# Autodesk Inventor assembly: A2017_T4_11
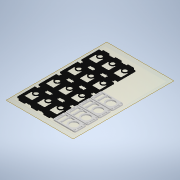
[picture p0: Inventor's stored thumbnail of the model, 180x180]
Saved by Autodesk Inventor 2020 (Build 240168000, 168)
## iProperties
Created: 2021-08-27
Part Number: A2017_T4_11
Document SubType Name: Assembly
Designer: Masato
Author: Masato
## Documents named in this file (4)
- C:\Inventor\SUSTAINA-OP\Cam\A2017_T4_11.iam
- C:\Inventor\SUSTAINA-OP\Cam\DisposableBoard.ipt
- C:\Inventor\SUSTAINA-OP\UpperBody\Trunk\Trunk_neck_frame.ipt
- C:\Inventor\SUSTAINA-OP\UpperBody\Trunk\Trunk_servo_bottom_frame.ipt
## Components (23 placed, 3 different names)
1. DisposableBoard:1 — メイト:2, メイト:1, フラッシュ:1, フラッシュ:2, メイト:8, フラッシュ:5, フラッシュ:6, メイト:10
2. Trunk_neck_frame:2 — メイト:10, フラッシュ:7, メイト:11
3. Trunk_neck_frame:3
4. Trunk_neck_frame:4
5. Trunk_neck_frame:5
6. Trunk_servo_bottom_frame:1 — メイト:8, フラッシュ:5, フラッシュ:6, フラッシュ:7
7. Trunk_servo_bottom_frame:2
8. Trunk_servo_bottom_frame:3 — メイト:11
9. Trunk_servo_bottom_frame:4
10. Trunk_servo_bottom_frame:5
11. Trunk_servo_bottom_frame:6
12. Trunk_servo_bottom_frame:7
13. Trunk_servo_bottom_frame:8
14. Trunk_servo_bottom_frame:9
15. Trunk_servo_bottom_frame:10
16. Trunk_servo_bottom_frame:11
17. Trunk_servo_bottom_frame:12
18. Trunk_servo_bottom_frame:13
19. Trunk_servo_bottom_frame:14
20. Trunk_servo_bottom_frame:15
21. Trunk_servo_bottom_frame:16
22. Trunk_servo_bottom_frame:17
23. Trunk_servo_bottom_frame:18
## Component patterns: (2 elements), (3 elements), (2 elements, first: Trunk_neck_frame:2), コンポーネント パターン 3:2 (2 elements), (2 elements), コンポーネント パターン 4:2 (2 elements), コンポーネント パターン 4:3 (2 elements), (3 elements, first: Trunk_servo_bottom_frame:1), コンポーネント パターン 2:2 (3 elements), コンポーネント パターン 2:3 (3 elements), コンポーネント パターン 2:4 (3 elements), コンポーネント パターン 2:5 (3 elements), コンポーネント パターン 2:6 (3 elements)
## Relationships (10: Mate 5, Flush 5)
- メイト:2 [Mate]: DisposableBoard:1
- メイト:1 [Mate]: DisposableBoard:1
- フラッシュ:1 [Flush]: DisposableBoard:1
- フラッシュ:2 [Flush]: DisposableBoard:1
- メイト:8 [Mate]: DisposableBoard:1 ↔ Trunk_servo_bottom_frame:1
- フラッシュ:5 [Flush] (5 mm): DisposableBoard:1 ↔ Trunk_servo_bottom_frame:1
- フラッシュ:6 [Flush] (2 mm): DisposableBoard:1 ↔ Trunk_servo_bottom_frame:1
- メイト:10 [Mate]: DisposableBoard:1 ↔ Trunk_neck_frame:2
- フラッシュ:7 [Flush]: Trunk_neck_frame:2 ↔ Trunk_servo_bottom_frame:1
- メイト:11 [Mate] (2.5 mm): Trunk_neck_frame:2 ↔ Trunk_servo_bottom_frame:3
